# Autodesk Inventor assembly: KAKI
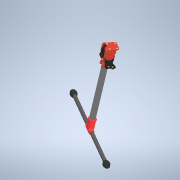
[picture p0: Inventor's stored thumbnail of the model, 180x180]
Saved by Autodesk Inventor 2020 (Build 240168000, 168)
## iProperties
Created: 2020-03-27
Part Number: KAKI
Document SubType Name: Assembly
Designer: Muhyidin
Author: Muhyidin
## Documents named in this file (8)
- D:\ITS\BAYUCARAKA\PROYEK '19\IKI\KAKI.iam
- D:\ITS\BAYUCARAKA\PROYEK '19\IKI\20021-007,008,009_leg-pivot v11.iam
- D:\ITS\BAYUCARAKA\PROYEK '19\IKI\20021-004_arm-pivot v7.iam
- D:\ITS\BAYUCARAKA\PROYEK '19\IKI\20021-010_leg v2.ipt
- D:\ITS\BAYUCARAKA\PROYEK '19\IKI\20021-003_arm-clip v7.iam
- D:\ITS\BAYUCARAKA\PROYEK '19\IKI\20021-011_landing-gear-connector v3.ipt
- D:\ITS\BAYUCARAKA\PROYEK '19\IKI\20021-012_small-tube v3.ipt
- D:\ITS\BAYUCARAKA\PROYEK '19\IKI\20021-013_landing-gear-foot v3.ipt
## Components (8 placed, 7 different names)
1. 20021-007,008,009_leg-pivot v11:2 [sub-assembly] — Rotational:27, Rotational:32
2. 20021-004_arm-pivot v7:1 [sub-assembly] — Rotational:27, Rotational:30
3. 20021-010_leg v2:1 — Rotational:30, Rotational:33
4. 20021-003_arm-clip v7:1 [sub-assembly] — Rotational:32
5. 20021-011_landing-gear-connector v3:1 — Rotational:33, Cylindrical:1
6. 20021-012_small-tube v3:1 — Cylindrical:1, Rigid:2, Rotational:37
7. 20021-013_landing-gear-foot v3:3 — Rigid:2
8. 20021-013_landing-gear-foot v3:4 — Rotational:37
## Relationships (7: RevoluteJoint 5, CylindricalJoint 1, WeldJoint 1)
- Rotational:27 [RevoluteJoint]: 20021-007,008,009_leg-pivot v11:2 ↔ 20021-004_arm-pivot v7:1
- Rotational:30 [RevoluteJoint]: 20021-004_arm-pivot v7:1 ↔ 20021-010_leg v2:1
- Rotational:32 [RevoluteJoint]: 20021-007,008,009_leg-pivot v11:2 ↔ 20021-003_arm-clip v7:1
- Rotational:33 [RevoluteJoint]: 20021-010_leg v2:1 ↔ 20021-011_landing-gear-connector v3:1
- Cylindrical:1: 20021-011_landing-gear-connector v3:1 ↔ 20021-012_small-tube v3:1
- Rigid:2 [WeldJoint]: 20021-012_small-tube v3:1 ↔ 20021-013_landing-gear-foot v3:3
- Rotational:37 [RevoluteJoint]: 20021-012_small-tube v3:1 ↔ 20021-013_landing-gear-foot v3:4
